# Autodesk Inventor assembly: Frame
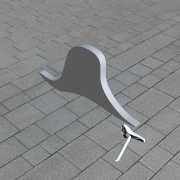
[picture p0: Inventor's stored thumbnail of the model, 180x180]
Saved by Autodesk Inventor 2014 (Build 180170000, 170)
## iProperties
Created: 2015-03-25
Part Number: Frame
Document SubType Name: Assembly
Designer: Yann
Author: Yann
## Documents named in this file (3)
- C:\Users\Yann\Documents\GitHub\BIKAIR_CAD\Source\Frame\Frame.iam
- C:\Users\Yann\Documents\GitHub\BIKAIR_CAD\Source\Frame\Frame_Generator.ipt
- C:\Users\Yann\Documents\GitHub\BIKAIR_CAD\Source\Frame\Seat.iam
## Components (2 placed, 2 different names)
1. Frame_Generator:1 — Affleurement:2, Placage:1, Placage:2
2. Seat:1 [sub-assembly]
## Relationships (3: Mate 2, Flush 1)
- Affleurement:2 [Flush]: Frame_Generator:1
- Placage:1 [Mate]: Frame_Generator:1
- Placage:2 [Mate]: Frame_Generator:1
